# Autodesk Inventor assembly: Pièce 22-24-120x70
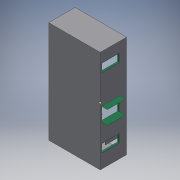
[picture p0: Inventor's stored thumbnail of the model, 180x180]
Saved by Autodesk Inventor 2016 SP1 (Build 200210100, 210)
## iProperties
Created: 2016-10-04
Part Number: Pièce 22-24-120x70
Material: Générique
Document SubType Name: Assembly
Designer: dimercur
Author: dimercur
## Documents named in this file (8)
- D:\Users\dimercur\Documents\SVN\projets-gei\Salle 22-24\Pièce 22-24-120x70.iam
- D:\Users\dimercur\Documents\SVN\projets-gei\Salle 22-24\Pièce.ipt
- D:\Users\dimercur\Documents\SVN\projets-gei\Salle 22-24\Fenetre.iam
- D:\Users\dimercur\Documents\SVN\projets-gei\Salle 22-24\Porte Simple.ipt
- D:\Users\dimercur\Documents\SVN\projets-gei\Salle 22-24\Porte Double.ipt
- D:\Users\dimercur\Documents\SVN\projets-gei\Salle 22-24\Couvre-Radiateur.ipt
- D:\Users\dimercur\Documents\SVN\projets-gei\Salle 22-24\Ecran_Videoprojecteur.ipt
- D:\Users\dimercur\Documents\SVN\projets-gei\Salle 22-24\Poste de Travail - Quetzal.iam
## Components (44 placed, 7 different names)
1. Pièce:1 — Placage:1, Placage:2, Placage:3, Placage:4, Placage:5, Placage:6, Placage:7, Placage:8, Placage:9, Placage:10, Placage:14, Placage:15, Placage:16, Placage:17, Placage:18, Affleurement:1, Placage:19, Placage:20, Placage:21, Placage:22, Placage:23, Placage:24, Placage:25, Placage:26, Placage:28, Placage:30
2. Porte Simple:1 — Placage:5, Placage:6, Placage:9
3. Porte Double:1 — Placage:4, Placage:7, Placage:8
4. Couvre-Radiateur:1 — Placage:14, Placage:15, Placage:16, Placage:27, Placage:32
5. Porte Simple:2 — Placage:17, Placage:18, Affleurement:1
6. Ecran_Videoprojecteur:1 — Placage:20, Placage:22, Placage:23
7. Ecran_Videoprojecteur:2 — Placage:19, Placage:21, Placage:24
8. Fenetre:1 [sub-assembly] — Placage:1, Placage:2, Placage:3
9. Fenetre:2 [sub-assembly]
10. Fenetre:3 [sub-assembly]
11. Fenetre:4 [sub-assembly]
12. Fenetre:5 [sub-assembly]
13. Fenetre:6 [sub-assembly]
14. Fenetre:7 [sub-assembly]
15. Poste de Travail - Quetzal:23 [sub-assembly] — Placage:30, Placage:31, Placage:32
16. Poste de Travail - Quetzal:24 [sub-assembly]
17. Poste de Travail - Quetzal:25 [sub-assembly]
18. Poste de Travail - Quetzal:26 [sub-assembly]
19. Poste de Travail - Quetzal:27 [sub-assembly]
20. Poste de Travail - Quetzal:28 [sub-assembly]
21. Poste de Travail - Quetzal:29 [sub-assembly]
22. Poste de Travail - Quetzal:30 [sub-assembly]
23. Poste de Travail - Quetzal:1 [sub-assembly] — Placage:25, Placage:27, Placage:28, Placage:29
24. Poste de Travail - Quetzal:3 [sub-assembly]
25. Poste de Travail - Quetzal:4 [sub-assembly]
26. Poste de Travail - Quetzal:5 [sub-assembly] — Affleurement:2
27. Poste de Travail - Quetzal:8 [sub-assembly]
28. Poste de Travail - Quetzal:9 [sub-assembly]
29. Poste de Travail - Quetzal:10 [sub-assembly]
30. Poste de Travail - Quetzal:11 [sub-assembly]
31. Poste de Travail - Quetzal:12 [sub-assembly]
32. Poste de Travail - Quetzal:13 [sub-assembly] — Placage:31
33. Poste de Travail - Quetzal:14 [sub-assembly]
34. Poste de Travail - Quetzal:15 [sub-assembly]
35. Poste de Travail - Quetzal:16 [sub-assembly]
36. Poste de Travail - Quetzal:17 [sub-assembly]
37. Poste de Travail - Quetzal:18 [sub-assembly]
38. Poste de Travail - Quetzal:19 [sub-assembly]
39. Poste de Travail - Quetzal:2 [sub-assembly] — Placage:26, Placage:29, Affleurement:2
40. Poste de Travail - Quetzal:6 [sub-assembly]
41. Poste de Travail - Quetzal:7 [sub-assembly]
42. Poste de Travail - Quetzal:20 [sub-assembly]
43. Poste de Travail - Quetzal:21 [sub-assembly]
44. Poste de Travail - Quetzal:22 [sub-assembly]
## Component patterns: (7 elements, first: Fenetre:1), (4 elements), (2 elements), (8 elements, first: Poste de Travail - Quetzal:23), (4 elements, first: Poste de Travail - Quetzal:1), Réseau de composants 5:2 (4 elements), Réseau de composants 5:3 (4 elements), Réseau de composants 5:4 (4 elements), (3 elements, first: Poste de Travail - Quetzal:2), Réseau de composants 6:2 (3 elements)
## Relationships (31: Mate 29, Flush 2)
- Placage:1 [Mate]: Pièce:1 ↔ Fenetre:1
- Placage:2 [Mate]: Pièce:1 ↔ Fenetre:1
- Placage:3 [Mate] (100 mm): Pièce:1 ↔ Fenetre:1
- Placage:4 [Mate]: Pièce:1 ↔ Porte Double:1
- Placage:5 [Mate]: Pièce:1 ↔ Porte Simple:1
- Placage:6 [Mate]: Pièce:1 ↔ Porte Simple:1
- Placage:7 [Mate]: Pièce:1 ↔ Porte Double:1
- Placage:8 [Mate]: Pièce:1 ↔ Porte Double:1
- Placage:9 [Mate]: Pièce:1 ↔ Porte Simple:1
- Placage:10 [Mate]: Pièce:1
- Placage:14 [Mate]: Pièce:1 ↔ Couvre-Radiateur:1
- Placage:15 [Mate]: Pièce:1 ↔ Couvre-Radiateur:1
- Placage:16 [Mate] (760 mm): Pièce:1 ↔ Couvre-Radiateur:1
- Placage:17 [Mate]: Pièce:1 ↔ Porte Simple:2
- Placage:18 [Mate]: Pièce:1 ↔ Porte Simple:2
- Affleurement:1 [Flush]: Pièce:1 ↔ Porte Simple:2
- Placage:19 [Mate]: Pièce:1 ↔ Ecran_Videoprojecteur:2
- Placage:20 [Mate]: Pièce:1 ↔ Ecran_Videoprojecteur:1
- Placage:21 [Mate] (700 mm): Pièce:1 ↔ Ecran_Videoprojecteur:2
- Placage:22 [Mate] (700 mm): Pièce:1 ↔ Ecran_Videoprojecteur:1
- Placage:23 [Mate] (1800 mm): Pièce:1 ↔ Ecran_Videoprojecteur:1
- Placage:24 [Mate] (2700 mm): Pièce:1 ↔ Ecran_Videoprojecteur:2
- Placage:25 [Mate]: Pièce:1 ↔ Poste de Travail - Quetzal:1
- Placage:26 [Mate]: Pièce:1 ↔ Poste de Travail - Quetzal:2
- Placage:27 [Mate]: Couvre-Radiateur:1 ↔ Poste de Travail - Quetzal:1
- Placage:28 [Mate]: Pièce:1 ↔ Poste de Travail - Quetzal:1
- Placage:29 [Mate]: Poste de Travail - Quetzal:1 ↔ Poste de Travail - Quetzal:2
- Affleurement:2 [Flush]: Poste de Travail - Quetzal:5 ↔ Poste de Travail - Quetzal:2
- Placage:30 [Mate]: Pièce:1 ↔ Poste de Travail - Quetzal:23
- Placage:31 [Mate]: Poste de Travail - Quetzal:23 ↔ Poste de Travail - Quetzal:13
- Placage:32 [Mate]: Couvre-Radiateur:1 ↔ Poste de Travail - Quetzal:23
